# Autodesk Inventor assembly: WheelGear
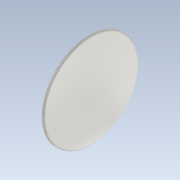
[picture p0: Inventor's stored thumbnail of the model, 180x180]
Saved by Autodesk Inventor 2021 (Build 250183000, 183)
## iProperties
Created: 2021-08-29
Part Number: WheelGear
Document SubType Name: Assembly
Designer: digge
Author: digge
## Documents named in this file (2)
- C:\Users\digge\Documents\Inventor\Projects\FerrisWheel\WheelGear.iam
- C:\Users\digge\Documents\Inventor\Projects\FerrisWheel\WheelGear\Design Accelerator\Spur Gears1.iam
## Components (1 placed, 1 different names)
1. Spur Gears:1 [sub-assembly]
## Named parameters: ScrewWidth = 3 mm
